# Autodesk Inventor assembly: Collumn
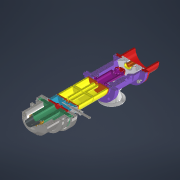
[picture p0: Inventor's stored thumbnail of the model, 180x180]
Saved by Autodesk Inventor 2022 (Build 260153000, 153)
## iProperties
Created: 2022-03-30
Part Number: Collumn
Document SubType Name: Assembly
Designer: Vinicius Miguel
Author: Vinicius Miguel
## Documents named in this file (8)
- C:\ViniFiles\SEM-Mechanical\Collumn.iam
- C:\ViniFiles\SEM-Mechanical\Objective.iam
- C:\ViniFiles\SEM-Mechanical\Condensers.iam
- C:\ViniFiles\SEM-Mechanical\008.ipt
- C:\ViniFiles\SEM-Mechanical\Anode.iam
- C:\ViniFiles\SEM-Mechanical\ElectronGun.iam
- C:\ViniFiles\SEM-Mechanical\022.ipt
- C:\ViniFiles\SEM-Mechanical\023.ipt
## Components (7 placed, 7 different names)
1. Objective:1 [sub-assembly] — Mate:1, Flush:1, Flush:2, Mate:4, Mate:10
2. Condensers:1 [sub-assembly] — Mate:2, Mate:5, Mate:9
3. 008:1 — Mate:3, Mate:4, Mate:5, Mate:6, Mate:11, Mate:13, Mate:14, Mate:15
4. Anode:1 [sub-assembly] — Mate:7, Mate:9, Rotational:1, Mate:10, Mate:16
5. ElectronGun:1 [sub-assembly] — Rotational:1, Mate:16
6. 022:1 — Mate:11, Mate:12, Mate:14, Mate:15
7. 023:1 — Mate:12, Mate:13
## Relationships (18: Mate 15, Flush 2, RevoluteJoint 1)
- Mate:1: Objective:1
- Flush:1: Objective:1
- Flush:2: Objective:1
- Mate:2: Condensers:1
- Mate:3: 008:1
- Mate:4: Objective:1 ↔ 008:1
- Mate:5: Condensers:1 ↔ 008:1
- Mate:6: 008:1
- Mate:7: Anode:1
- Mate:9: Condensers:1 ↔ Anode:1
- Rotational:1 [RevoluteJoint]: Anode:1 ↔ ElectronGun:1
- Mate:10: Objective:1 ↔ Anode:1
- Mate:11: 008:1 ↔ 022:1
- Mate:12: 022:1 ↔ 023:1
- Mate:13: 008:1 ↔ 023:1
- Mate:14: 008:1 ↔ 022:1
- Mate:15: 008:1 ↔ 022:1
- Mate:16: Anode:1 ↔ ElectronGun:1
